# Autodesk Inventor assembly: 2200_Coil Housing
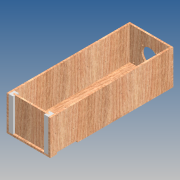
[picture p0: Inventor's stored thumbnail of the model, 180x180]
Saved by Autodesk Inventor 2020 (Build 240168000, 168)
## iProperties
Created: 2019-11-08
Part Number: 2200_Coil Housing
Document SubType Name: Assembly
Designer: RFLab
Author: RFLab
## Documents named in this file (6)
- C:\Users\RFLab\Dropbox\MPI Group Folder\MPS\Inventor_Parts\Parts Numbered - OSMPI\2xxx_Sample Holder and Rx\22xx_Coil Housing\2200_Coil Housing.iam
- C:\Users\RFLab\Dropbox\MPI Group Folder\MPS\Inventor_Parts\MPS System Assembly\V2\2019_11_08_box_part1_front.ipt
- C:\Users\RFLab\Dropbox\MPI Group Folder\MPS\Inventor_Parts\MPS System Assembly\V2\2019_11_08_box_part2.ipt
- C:\Users\RFLab\Dropbox\MPI Group Folder\MPS\Inventor_Parts\MPS System Assembly\V2\2019_11_08_box_part3.ipt
- C:\Users\RFLab\Dropbox\MPI Group Folder\MPS\Inventor_Parts\MPS System Assembly\V2\2019_11_18_box_part1_back_without_holes.ipt
- C:\Users\RFLab\Dropbox\MPI Group Folder\MPS\Inventor_Parts\MPS System Assembly\V2\2020_01_15_holder_box.ipt
## Components (7 placed, 5 different names)
1. 2019_11_08_box_part1_front:1 — Flush:1, Mate:3, Mate:4, Flush:2, Mate:9, Flush:17
2. 2019_11_08_box_part2:1 — Flush:1, Flush:11, Mate:9, Mate:10, Flush:13, Mate:13, Flush:15
3. 2019_11_08_box_part2:2 — Mate:3, Mate:4, Flush:2, Mate:8, Flush:10, Mate:12, Flush:12, Flush:14, Flush:16
4. 2019_11_08_box_part3:1 — Mate:8, Flush:10, Flush:11, Mate:10, Mate:11, Flush:17
5. 2019_11_18_box_part1_back_without_holes:1 — Mate:11, Mate:14, Flush:16, Mate:15
6. 2020_01_15_holder_box:1 — Mate:12, Flush:12, Flush:14, Mate:14, Mate:15
7. 2020_01_15_holder_box:2 — Flush:13, Mate:13, Flush:15
## Relationships (20: Flush 10, Mate 10)
- Flush:1: 2019_11_08_box_part1_front:1 ↔ 2019_11_08_box_part2:1
- Mate:3: 2019_11_08_box_part1_front:1 ↔ 2019_11_08_box_part2:2
- Mate:4: 2019_11_08_box_part1_front:1 ↔ 2019_11_08_box_part2:2
- Flush:2: 2019_11_08_box_part1_front:1 ↔ 2019_11_08_box_part2:2
- Mate:8: 2019_11_08_box_part2:2 ↔ 2019_11_08_box_part3:1
- Flush:10: 2019_11_08_box_part2:2 ↔ 2019_11_08_box_part3:1
- Flush:11: 2019_11_08_box_part2:1 ↔ 2019_11_08_box_part3:1
- Mate:9: 2019_11_08_box_part1_front:1 ↔ 2019_11_08_box_part2:1
- Mate:10: 2019_11_08_box_part2:1 ↔ 2019_11_08_box_part3:1
- Mate:11: 2019_11_08_box_part3:1 ↔ 2019_11_18_box_part1_back_without_holes:1
- Mate:12: 2019_11_08_box_part2:2 ↔ 2020_01_15_holder_box:1
- Flush:12: 2019_11_08_box_part2:2 ↔ 2020_01_15_holder_box:1
- Flush:13: 2019_11_08_box_part2:1 ↔ 2020_01_15_holder_box:2
- Mate:13: 2019_11_08_box_part2:1 ↔ 2020_01_15_holder_box:2
- Flush:14: 2019_11_08_box_part2:2 ↔ 2020_01_15_holder_box:1
- Flush:15: 2019_11_08_box_part2:1 ↔ 2020_01_15_holder_box:2
- Mate:14: 2019_11_18_box_part1_back_without_holes:1 ↔ 2020_01_15_holder_box:1
- Flush:16: 2019_11_08_box_part2:2 ↔ 2019_11_18_box_part1_back_without_holes:1
- Mate:15: 2019_11_18_box_part1_back_without_holes:1 ↔ 2020_01_15_holder_box:1
- Flush:17: 2019_11_08_box_part1_front:1 ↔ 2019_11_08_box_part3:1
